# Autodesk Inventor assembly: Toughbox-mini
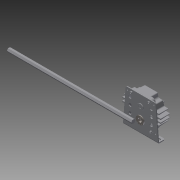
[picture p0: Inventor's stored thumbnail of the model, 180x180]
Saved by Autodesk Inventor 2015 SP1 (Build 190203100, 203)
## iProperties
Created: 2015-01-17
Part Number: Toughbox-mini
Document SubType Name: Assembly
Designer: Jarod
Author: Unknown
Title: S:/Products/Gearboxes Spur Single Stage/Toughbox/Toughbox Mini/Toughbox-Mini.stp
Organization: Unknown
Description: Unknown
Sending System: Unknown
Preprocessor: XStep 1.0
Author: Jarod
## Documents named in this file (16)
- C:\Users\Jarod\Documents\Westview\Robotics\FRC\2015\CAD\Robot\Chassis\Imported Components\Toughbox-mini\Toughbox-mini.iam
- C:\Users\Jarod\Documents\Westview\Robotics\FRC\2015\CAD\Robot\Chassis\Imported Components\Toughbox-mini\r6zz.ipt
- C:\Users\Jarod\Documents\Westview\Robotics\FRC\2015\CAD\Robot\Chassis\Imported Components\Toughbox-mini\Toughbox_d07.ipt
- C:\Users\Jarod\Documents\Westview\Robotics\FRC\2015\CAD\Robot\Chassis\Imported Components\Toughbox-mini\Toughbox_d05.ipt
- C:\Users\Jarod\Documents\Westview\Robotics\FRC\2015\CAD\Robot\Chassis\Imported Components\Toughbox-mini\Toughbox_d08.ipt
- C:\Users\Jarod\Documents\Westview\Robotics\FRC\2015\CAD\Robot\Chassis\Imported Components\Toughbox-mini\Toughbox_d06.ipt
- C:\Users\Jarod\Documents\Westview\Robotics\FRC\2015\CAD\Robot\Chassis\Imported Components\Toughbox-mini\fr-6-zz.ipt
- C:\Users\Jarod\Documents\Westview\Robotics\FRC\2015\CAD\Robot\Chassis\Imported Components\Toughbox-mini\10-32_nylock_nut.ipt
- C:\Users\Jarod\Documents\Westview\Robotics\FRC\2015\CAD\Robot\Chassis\Imported Components\Toughbox-mini\5-16_washer.ipt
- C:\Users\Jarod\Documents\Westview\Robotics\FRC\2015\CAD\Robot\Chassis\Imported Components\Toughbox-mini\Toughbox_d09.ipt
- C:\Users\Jarod\Documents\Westview\Robotics\FRC\2015\CAD\Robot\Chassis\Imported Components\Toughbox-mini\8mm_spring_clip.ipt
- C:\Users\Jarod\Documents\Westview\Robotics\FRC\2015\CAD\Robot\Chassis\Imported Components\Toughbox-mini\Toughbox-mini_d01-5-12.ipt
- C:\Users\Jarod\Documents\Westview\Robotics\FRC\2015\CAD\Robot\Chassis\Imported Components\Toughbox-mini\Toughbox-mini_d02.ipt
- C:\Users\Jarod\Documents\Westview\Robotics\FRC\2015\CAD\Robot\Chassis\Imported Components\Toughbox-mini\10-32x0625_shcs.ipt
- C:\Users\Jarod\Documents\Westview\Robotics\FRC\2015\CAD\Robot\Chassis\Imported Components\0.5 Hex Bearing\0.5 Hex Bearing.ipt
- C:\Users\Jarod\Documents\Westview\Robotics\FRC\2015\CAD\Robot\Chassis\0.5 hex output shaft.ipt
## Components (31 placed, 15 different names)
1. r6zz
2. r6zz:1 — Mate:3
3. Toughbox_d07
4. Toughbox_d05
5. Toughbox_d08
6. Toughbox_d06
7. fr-6-zz
8. 10-32_nylock_nut
9. 10-32_nylock_nut:1
10. 10-32_nylock_nut:2
11. 10-32_nylock_nut:3
12. 5-16_washer
13. 5-16_washer:1
14. 5-16_washer:2
15. 5-16_washer:3
16. Toughbox_d09
17. Toughbox_d09:1
18. 8mm_spring_clip
19. 8mm_spring_clip:1
20. Toughbox-mini_d01-5-12
21. Toughbox-mini_d02 — Mate:1, Mate:2
22. 10-32x0625_shcs
23. 10-32x0625_shcs:1
24. 10-32x0625_shcs:2
25. 10-32x0625_shcs:3
26. 10-32x0625_shcs:4
27. 10-32x0625_shcs:5
28. 10-32x0625_shcs:6
29. 10-32x0625_shcs:7
30. 0.5 Hex Bearing:1 — Mate:1, Mate:2, Mate:4, Mate:5
31. 0.5 hex output shaft:1 — Mate:3, Mate:4, Mate:5
## Relationships (5: Mate 5)
- Mate:1: Toughbox-mini_d02 ↔ 0.5 Hex Bearing:1
- Mate:2: Toughbox-mini_d02 ↔ 0.5 Hex Bearing:1
- Mate:3: r6zz:1 ↔ 0.5 hex output shaft:1
- Mate:4: 0.5 Hex Bearing:1 ↔ 0.5 hex output shaft:1
- Mate:5: 0.5 Hex Bearing:1 ↔ 0.5 hex output shaft:1
